# Autodesk Inventor assembly: Tubo auxiliar 1
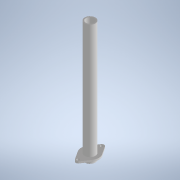
[picture p0: Inventor's stored thumbnail of the model, 180x180]
Saved by Autodesk Inventor 2021 (Build 250183000, 183)
## iProperties
Created: 2021-07-23
Part Number: Tubo auxiliar 1
Document SubType Name: Assembly
Designer: Giovanni
Author: Giovanni
## Documents named in this file (3)
- C:\Users\irineu\Documents\Inventor\MotorRadial7\Tubo auxiliar 1.iam
- C:\Users\irineu\Documents\Inventor\MotorRadial7\Peça27.ipt
- C:\Users\irineu\Documents\Inventor\MotorRadial7\Peça26.ipt
## Components (2 placed, 2 different names)
1. Peça27:1 — Coincidente:2, Inserir:1
2. Peça26:1 — Inserir:1
## Relationships (2: Mate 1, Insert 1)
- Coincidente:2 [Mate]: Peça27:1
- Inserir:1 (-10 mm): Peça27:1 ↔ Peça26:1
